# Autodesk Inventor assembly: PIHTI-for-Boron_2026_non-bellows
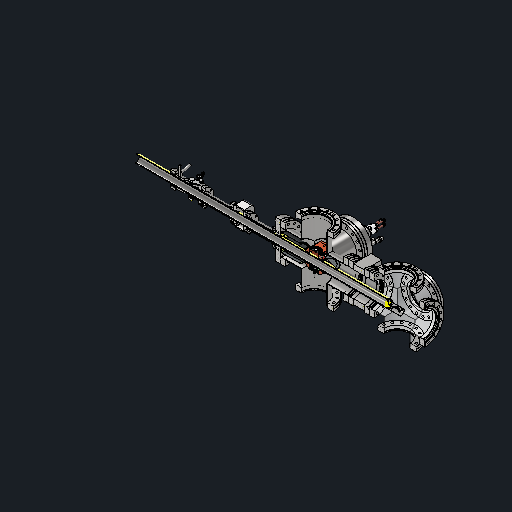
[picture p0: Inventor's stored thumbnail of the model, 512x512]
Saved by Autodesk Inventor 2027.1 (Build 311270010, 270A)
## iProperties
Created: 2024-05-09
Part Number: PIHTI-for-Boron_2026_non-bellows
Document SubType Name: Assembly
Designer: kuzmin
Mass: 19614.5 g
Surface Area: 13609.5 cm^2
Volume: 3689.47 cm^3
Density: 5.31636 g/cm^3
Author: kuzmin
## Documents named in this file (23)
- C:\Users\queezz\Dropbox\Drawings\pihti-cad\Plasma Vessel_2026\PIHTI-for-Boron_2026_non-bellows.iam
- C:\Users\queezz\Dropbox\Drawings\pihti-cad\Plasma Vessel\Plasma-vacuum-cross\Plasma-vacuum-vessel-152IC-cross.iam
- C:\Users\queezz\Dropbox\Drawings\pihti-cad\Plasma Vessel\Plasma-Box\Plasma-box-hayashi-aka-upgrade.iam
- C:\Users\queezz\Dropbox\Drawings\pihti-cad\ContentCenter\Fastners\M3x8-SHCS.ipt
- C:\Users\queezz\Dropbox\Drawings\pihti-cad\Plasma Vessel\Plasma-Box\probe-gate-with-spindel.iam
- C:\Users\queezz\Dropbox\Drawings\pihti-cad\Plasma Vessel\Cathode-Anode-Flange\cf70_spacer.ipt
- C:\Users\queezz\Dropbox\Drawings\pihti-cad\Plasma Vessel\entrance-mesh-assembly.iam
- C:\Users\queezz\Dropbox\Drawings\pihti-cad\Plasma Vessel\probe-port-mesh-welded.iam
- C:\Users\queezz\Dropbox\Drawings\pihti-cad\ContentCenter\CF-parts\CF70-nipple\CF70-nipple.iam
- C:\Users\queezz\Dropbox\Drawings\pihti-cad\ContentCenter\CF-parts\CF70-gate-valve\Gatevalve_70_pneumatic.iam
- C:\Users\queezz\Dropbox\Drawings\pihti-cad\Plasma Vessel_2026\gate_valve\CF150-gatevalve-assembly.iam
- C:\Users\queezz\Dropbox\Drawings\pihti-cad\Plasma Vessel_2026\Plasma-vacuum-vessel\Plasma-vacuum-vessel-152IC-cross-L205p8.iam
- C:\Users\queezz\Dropbox\Drawings\pihti-cad\ContentCenter\CF-parts\CF-70-Tee.ipt
- C:\Users\queezz\Dropbox\Drawings\pihti-cad\ContentCenter\CF-KF-adapters\ICF70_to_KF40.ipt
- C:\Users\queezz\Dropbox\Drawings\pihti-cad\Plasma Vessel\Cathode-Anode-Flange\Cathode-Anode-70IC-flange-with-feeds.iam
- C:\Users\queezz\Dropbox\Drawings\pihti-cad\Plasma Vessel\Plasma-Flange-2024\cathode-box-on-a-flange.iam
- C:\Users\queezz\Dropbox\Drawings\pihti-cad\ContentCenter\NW\NW40_viton_centering_ring.ipt
- C:\Users\queezz\Dropbox\Drawings\pihti-cad\ContentCenter\NW\NW40_clamp.ipt
- C:\Users\queezz\Dropbox\Drawings\pihti-cad\Plasma Vessel_2026\contents\CF_152-70_bearing.ipt
- C:\Users\queezz\Dropbox\Drawings\pihti-cad\BoronProbe_2026\parts\B_probe_bearing.ipt
- C:\Users\queezz\Dropbox\Drawings\pihti-cad\Plasma Vessel_2026\contents\M4×12-VentedHexBolt.ipt
- C:\Users\queezz\Dropbox\Drawings\pihti-cad\PALP\OringFixture.iam
- C:\Users\queezz\Dropbox\Drawings\pihti-cad\BoronProbe_2026\BoronProbe_2026_non-bellows.iam
## Components (31 placed, 22 different names)
1. Plasma-vacuum-vessel-152IC-cross:1 [sub-assembly] — Mate:1, Flush:1, Flush:2, Rigid:18, Mate:22, Mate:23, Mate:24, Mate:59, Mate:60
2. Plasma-box-hayashi-aka-upgrade:1 [sub-assembly] — Mate:3, Mate:4, Hinge Angle, Mate:13, Mate:17
3. probe-gate-with-spindel:1 [sub-assembly] — Mate:3, Mate:4, Hinge Angle
4. cf70_spacer:1 — Mate:61, Mate:62, Mate:63, Mate:64
5. entrance-mesh-assembly:1 [sub-assembly] — Mate:13, Mate:17, Mate:19
6. probe-port-mesh-welded:1 [sub-assembly] — Mate:19
7. CF_152-70_bearing:1 — Rigid:18, Rigid:21, Mate:72, Mate:73, Mate:74
8. CF70-nipple:1 [sub-assembly] — Rigid:21, Rigid:22
9. Gatevalve_70_pneumatic:1 [sub-assembly] — Rigid:22, Mate:47, Mate:48, Mate:49
10. CF150-gatevalve-assembly:1 [sub-assembly] — Mate:22, Mate:23, Mate:24, Mate:44, Mate:45, Mate:46
11. Plasma-vacuum-vessel-152IC-cross-L205p8:1 [sub-assembly] — Mate:44, Mate:45, Mate:46
12. CF-70-Tee:1 — Mate:47, Mate:48, Mate:49, Mate:50, Mate:51, Mate:52
13. ICF70_to_KF40:1 — Mate:50, Mate:51, Mate:52, Mate:67, Mate:68, Mate:70, Mate:71
14. Cathode-Anode-70IC-flange-with-feeds:1 [sub-assembly] — Mate:63, Mate:64
15. cathode-box-on-a-flange:1 [sub-assembly] — Mate:59, Mate:60, Mate:61, Mate:62
16. NW40_viton_centering_ring:1 — Mate:67, Mate:68, Mate:81, Mate:82
17. NW40_clamp:1 — Mate:70, Mate:71
18. B_probe_bearing:1 — Mate:72, Mate:73, Mate:74, Mate:75, Mate:76, Mate:77, Mate:78, Mate:79, Mate:80
19. M4×12-VentedHexBolt:1 — Mate:75, Mate:76
20. M4×12-VentedHexBolt:2 — Mate:77, Mate:78
21. M4×12-VentedHexBolt:3 — Mate:79, Mate:80
22. OringFixture:1 [sub-assembly] — Mate:81, Mate:82, Mate:83, Flush:3
23. BoronProbe_2026_non-bellows:1 [sub-assembly] — Mate:83, Flush:3
24. SS ISO 4762 M3 x 8:5
25. SS ISO 4762 M3 x 8:6
26. SS ISO 4762 M3 x 8:7
27. SS ISO 4762 M3 x 8:8
28. SS ISO 4762 M3 x 8:1
29. SS ISO 4762 M3 x 8:2
30. SS ISO 4762 M3 x 8:3
31. SS ISO 4762 M3 x 8:4
## Relationships (47: Mate 40, Flush 3, WeldJoint 3, Angle 1)
- Mate:1: Plasma-vacuum-vessel-152IC-cross:1
- Flush:1: Plasma-vacuum-vessel-152IC-cross:1
- Flush:2: Plasma-vacuum-vessel-152IC-cross:1
- Mate:3: Plasma-box-hayashi-aka-upgrade:1 ↔ probe-gate-with-spindel:1
- Mate:4: Plasma-box-hayashi-aka-upgrade:1 ↔ probe-gate-with-spindel:1
- Hinge Angle [Angle] (45 deg): Plasma-box-hayashi-aka-upgrade:1 ↔ probe-gate-with-spindel:1
- Mate:13: Plasma-box-hayashi-aka-upgrade:1 ↔ entrance-mesh-assembly:1
- Mate:17: Plasma-box-hayashi-aka-upgrade:1 ↔ entrance-mesh-assembly:1
- Mate:19: entrance-mesh-assembly:1 ↔ probe-port-mesh-welded:1
- Rigid:18 [WeldJoint]: Plasma-vacuum-vessel-152IC-cross:1 ↔ CF_152-70_bearing:1
- Rigid:21 [WeldJoint]: CF_152-70_bearing:1 ↔ CF70-nipple:1
- Rigid:22 [WeldJoint]: CF70-nipple:1 ↔ Gatevalve_70_pneumatic:1
- Mate:22: Plasma-vacuum-vessel-152IC-cross:1 ↔ CF150-gatevalve-assembly:1
- Mate:23: Plasma-vacuum-vessel-152IC-cross:1 ↔ CF150-gatevalve-assembly:1
- Mate:24: Plasma-vacuum-vessel-152IC-cross:1 ↔ CF150-gatevalve-assembly:1
- Mate:44: CF150-gatevalve-assembly:1 ↔ Plasma-vacuum-vessel-152IC-cross-L205p8:1
- Mate:45: CF150-gatevalve-assembly:1 ↔ Plasma-vacuum-vessel-152IC-cross-L205p8:1
- Mate:46: CF150-gatevalve-assembly:1 ↔ Plasma-vacuum-vessel-152IC-cross-L205p8:1
- Mate:47: Gatevalve_70_pneumatic:1 ↔ CF-70-Tee:1
- Mate:48: Gatevalve_70_pneumatic:1 ↔ CF-70-Tee:1
- Mate:49: Gatevalve_70_pneumatic:1 ↔ CF-70-Tee:1
- Mate:50: CF-70-Tee:1 ↔ ICF70_to_KF40:1
- Mate:51: CF-70-Tee:1 ↔ ICF70_to_KF40:1
- Mate:52: CF-70-Tee:1 ↔ ICF70_to_KF40:1
- Mate:59: Plasma-vacuum-vessel-152IC-cross:1 ↔ cathode-box-on-a-flange:1
- Mate:60: Plasma-vacuum-vessel-152IC-cross:1 ↔ cathode-box-on-a-flange:1
- Mate:61: cf70_spacer:1 ↔ cathode-box-on-a-flange:1
- Mate:62: cf70_spacer:1 ↔ cathode-box-on-a-flange:1
- Mate:63: cf70_spacer:1 ↔ Cathode-Anode-70IC-flange-with-feeds:1
- Mate:64: cf70_spacer:1 ↔ Cathode-Anode-70IC-flange-with-feeds:1
- Mate:67: ICF70_to_KF40:1 ↔ NW40_viton_centering_ring:1
- Mate:68: ICF70_to_KF40:1 ↔ NW40_viton_centering_ring:1
- Mate:70: ICF70_to_KF40:1 ↔ NW40_clamp:1
- Mate:71: ICF70_to_KF40:1 ↔ NW40_clamp:1
- Mate:72: CF_152-70_bearing:1 ↔ B_probe_bearing:1
- Mate:73: CF_152-70_bearing:1 ↔ B_probe_bearing:1
- Mate:74: CF_152-70_bearing:1 ↔ B_probe_bearing:1
- Mate:75: B_probe_bearing:1 ↔ M4×12-VentedHexBolt:1
- Mate:76: B_probe_bearing:1 ↔ M4×12-VentedHexBolt:1
- Mate:77: B_probe_bearing:1 ↔ M4×12-VentedHexBolt:2
- Mate:78: B_probe_bearing:1 ↔ M4×12-VentedHexBolt:2
- Mate:79: B_probe_bearing:1 ↔ M4×12-VentedHexBolt:3
- Mate:80: B_probe_bearing:1 ↔ M4×12-VentedHexBolt:3
- Mate:81: NW40_viton_centering_ring:1 ↔ OringFixture:1
- Mate:82: NW40_viton_centering_ring:1 ↔ OringFixture:1
- Mate:83: OringFixture:1 ↔ BoronProbe_2026_non-bellows:1
- Flush:3 (136 mm): OringFixture:1 ↔ BoronProbe_2026_non-bellows:1
## Named parameters: ProbePos = 136 mm, ProbePos_Max = 136 mm, ProbePos_Min = 462 mm, ProbePos_Ext = 1084 mm
